# Autodesk Inventor assembly: _TOP_Design
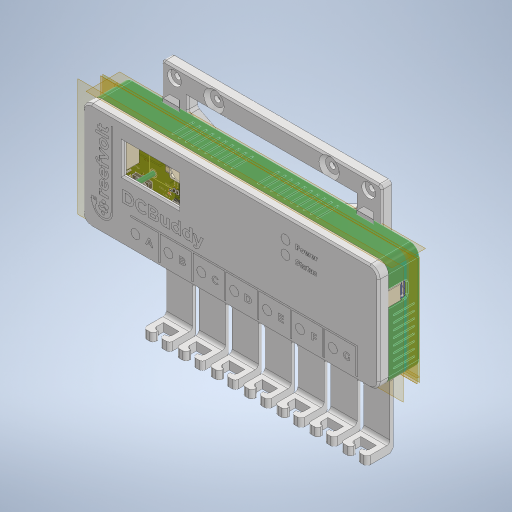
[picture p0: Inventor's stored thumbnail of the model, 512x512]
Saved by Autodesk Inventor 2024.3 (Build 283343000, 343)
## iProperties
Created: 2024-05-08
Part Number: _TOP_Design
Document SubType Name: Assembly
Designer: atrus
Author: atrus
## Documents named in this file (7)
- C:\Users\atrus\Dropbox\elec\Mechanical\DCBuddyV2\PCB\_TOP_Design.iam
- C:\Users\atrus\Dropbox\elec\Mechanical\DCBuddyV2\PCB\dcbuddy_v2.iam
- C:\Users\atrus\Dropbox\elec\Mechanical\DCBuddyV2\PCB\DCB2_BottomShell.ipt
- C:\Users\atrus\Dropbox\elec\Mechanical\DCBuddyV2\PCB\DCB2_TopShell.ipt
- C:\Users\atrus\Dropbox\elec\Mechanical\DCBuddyV2\OLED_With_Carrier.iam
- C:\Users\atrus\Dropbox\elec\Mechanical\DCBuddyV2\PCB\DCB2_Flange.ipt
- C:\Users\atrus\Dropbox\elec\Mechanical\DCBuddyV2\PCB\DCB2_CableClip.ipt
## Components (6 placed, 6 different names)
1. dcbuddy_v2:1 [sub-assembly] — Flush:1, Flush:2, Flush:6
2. DCB2_BottomShell:1 — Flush:1, Flush:2, Flush:3, Flush:4, Flush:6, Insert:1, Angle:1, Flush:7, Flush:8
3. DCB2_TopShell:1 — Flush:3, Flush:4
4. OLED_With_Carrier:1 [sub-assembly] — Insert:1, Angle:1
5. DCB2_Flange:1 — Flush:7, Flush:8, Flush:9, Flush:10
6. DCB2_CableClip:1 — Flush:9, Flush:10
## Relationships (11: Flush 9, Insert 1, Angle 1)
- Flush:1: dcbuddy_v2:1 ↔ DCB2_BottomShell:1
- Flush:2: dcbuddy_v2:1 ↔ DCB2_BottomShell:1
- Flush:3: DCB2_BottomShell:1 ↔ DCB2_TopShell:1
- Flush:4: DCB2_BottomShell:1 ↔ DCB2_TopShell:1
- Flush:6 (0.2032 mm): dcbuddy_v2:1 ↔ DCB2_BottomShell:1
- Insert:1 (-2.8 mm): DCB2_BottomShell:1 ↔ OLED_With_Carrier:1
- Angle:1 (90 deg): DCB2_BottomShell:1 ↔ OLED_With_Carrier:1
- Flush:7: DCB2_BottomShell:1 ↔ DCB2_Flange:1
- Flush:8: DCB2_BottomShell:1 ↔ DCB2_Flange:1
- Flush:9: DCB2_Flange:1 ↔ DCB2_CableClip:1
- Flush:10: DCB2_Flange:1 ↔ DCB2_CableClip:1
